# Autodesk Inventor assembly: Marco_apm_003-1
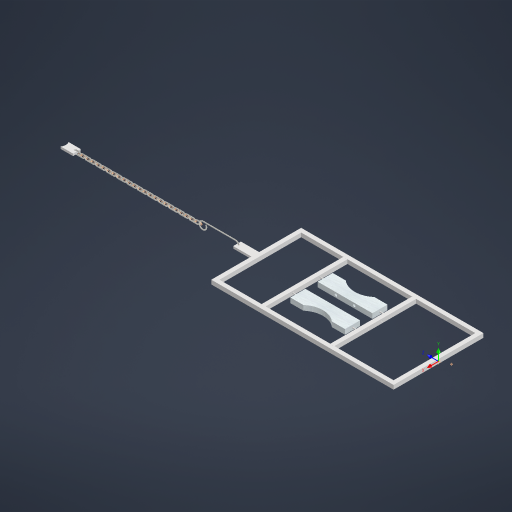
[picture p0: Inventor's stored thumbnail of the model, 512x512]
Saved by Autodesk Inventor 2024 (Build 280153000, 153)
## iProperties
Created: 2023-05-17
Part Number: Marco_apm_003-1
Document SubType Name: Assembly
Designer: javie
Author: javie
## Documents named in this file (6)
- C:\Users\javie\Downloads\Piezas CMR\Marco_APM_003\Marco_apm_003-1.iam
- C:\Users\javie\Downloads\Piezas CMR\Marco_Conveyor_Aereo.iam
- C:\Users\javie\Downloads\Piezas CMR\Marcos_solids\S_horizontal.ipt
- C:\Users\javie\Downloads\Piezas CMR\Marco_APM_003\Piezas\APM_003-1.ipt
- C:\Users\javie\Downloads\Piezas CMR\Marcos_solids\Topes_apm_2.ipt
- C:\Users\javie\Downloads\Piezas CMR\Marcos_solids\0111.ipt
## Components (8 placed, 5 different names)
1. Marco_Conveyor_Aereo:1 [sub-assembly] — Nivelación:1, Nivelación:2
2. S_horizontal:1 — Insertar:1, Insertar:2
3. APM_003-1:1 — Insertar:4, Insertar:7
4. APM_003-1:2 — Insertar:3, Insertar:8
5. Topes_apm_2:1 — Insertar:1, Insertar:2, Insertar:3, Insertar:4
6. S_horizontal:2 — Insertar:5, Insertar:6
7. Topes_apm_2:2 — Insertar:5, Insertar:6, Insertar:7, Insertar:8
8. 0111:1 — Nivelación:1, Nivelación:2
## Relationships (10: Insert 8, Flush 2)
- Insertar:1: S_horizontal:1 ↔ Topes_apm_2:1
- Insertar:2: S_horizontal:1 ↔ Topes_apm_2:1
- Insertar:3: APM_003-1:2 ↔ Topes_apm_2:1
- Insertar:4: APM_003-1:1 ↔ Topes_apm_2:1
- Insertar:5: S_horizontal:2 ↔ Topes_apm_2:2
- Insertar:6: S_horizontal:2 ↔ Topes_apm_2:2
- Insertar:7: APM_003-1:1 ↔ Topes_apm_2:2
- Insertar:8: APM_003-1:2 ↔ Topes_apm_2:2
- Nivelación:1 [Flush]: Marco_Conveyor_Aereo:1 ↔ 0111:1
- Nivelación:2 [Flush]: Marco_Conveyor_Aereo:1 ↔ 0111:1
